# Autodesk Inventor assembly: Moving Ramp Holder.ipt
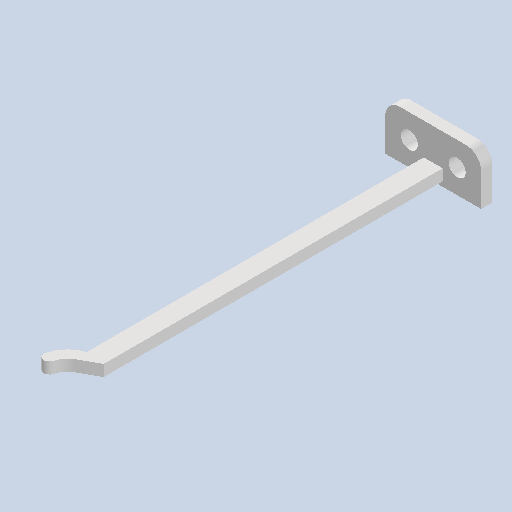
[picture p0: Inventor's stored thumbnail of the model, 512x512]
Saved by Autodesk Inventor 2025.1 (Build 291241020, 241B)
## iProperties
Created: 2024-10-27
Part Number: Moving Ramp Holder.ipt
Document SubType Name: Assembly
Designer: aly_g
Author: aly_g
## Documents named in this file (4)
- C:\Users\aly_g\Downloads\School\Eng Design\P1\CAD Model\Moving Ramp Holder.ipt.iam
- C:\Users\aly_g\Downloads\School\Eng Design\P1\CAD Model\Moving Ramp Holder Base.ipt
- C:\Users\aly_g\Downloads\School\Eng Design\P1\CAD Model\Moving Ramp Holder Shaft.ipt
- Moving Ramp Holder Shaft.ipt
## Components (2 placed, 2 different names)
1. Moving Ramp Holder Base:1 — Flush:1, Mate:1, Mate:2
2. Moving Ramp Holder Shaft:1 — Flush:1, Mate:1, Mate:2
## Relationships (3: Mate 2, Flush 1)
- Flush:1: Moving Ramp Holder Base:1 ↔ Moving Ramp Holder Shaft:1
- Mate:1: Moving Ramp Holder Base:1 ↔ Moving Ramp Holder Shaft:1
- Mate:2: Moving Ramp Holder Base:1 ↔ Moving Ramp Holder Shaft:1
